# Autodesk Inventor assembly: 尾翼
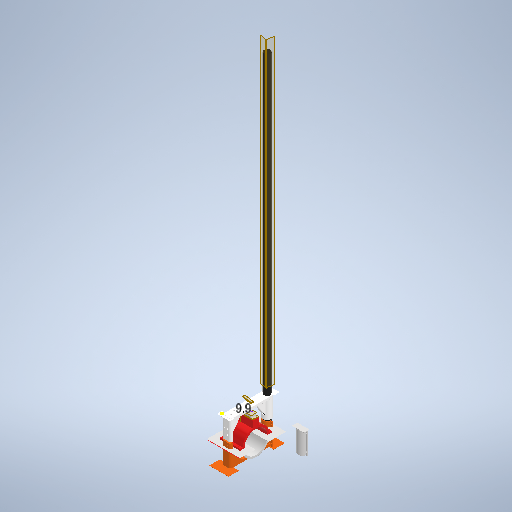
[picture p0: Inventor's stored thumbnail of the model, 512x512]
Saved by Autodesk Inventor 2025.2 (Build 292293000, 293)
## iProperties
Created: 2025-02-07
Part Number: 尾翼
Document SubType Name: Assembly
Designer: mahhy
Author: mahhy
## Documents named in this file (10)
- D:\兵庫県立大\鳥人間部\尾翼.iam
- D:\兵庫県立大\鳥人間部\motor-mount.ipt
- D:\兵庫県立大\鳥人間部\moror-mount1.ipt
- D:\兵庫県立大\鳥人間部\尾翼データ\servo_motor.ipt
- D:\兵庫県立大\鳥人間部\arm-1.ipt
- D:\兵庫県立大\鳥人間部\尾翼データ\wing1.ipt
- D:\兵庫県立大\鳥人間部\arm-2.ipt
- D:\兵庫県立大\鳥人間部\arm-2-2.ipt
- D:\兵庫県立大\鳥人間部\尾翼データ\bearing.ipt
- D:\兵庫県立大\鳥人間部\尾翼データ\pole.ipt
## Components (9 placed, 9 different names)
1. motor-mount:1 — リジッド:1, 挿入:6
2. moror-mount1:1 — リジッド:1, リジッド:2
3. servo_motor:1 — リジッド:2, 挿入:7
4. arm-1:1 — 挿入:7, メイト:1
5. wing1:1
6. arm-2:1 — 挿入:3, 挿入:5
7. arm-2-2:1
8. bearing:1 — 挿入:5, 挿入:6
9. pole:1 — 挿入:3, メイト:1
## Relationships (7: Insert 4, WeldJoint 2, Mate 1)
- リジッド:1 [WeldJoint]: motor-mount:1 ↔ moror-mount1:1
- リジッド:2 [WeldJoint]: moror-mount1:1 ↔ servo_motor:1
- 挿入:3 [Insert]: arm-2:1 ↔ pole:1
- 挿入:5 [Insert] (1 mm): arm-2:1 ↔ bearing:1
- 挿入:6 [Insert]: motor-mount:1 ↔ bearing:1
- 挿入:7 [Insert] (7 mm): servo_motor:1 ↔ arm-1:1
- メイト:1 [Mate]: arm-1:1 ↔ pole:1
